# Autodesk Inventor assembly: Cover
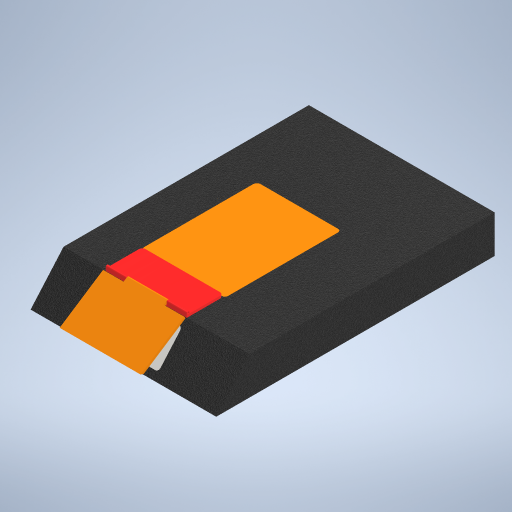
[picture p0: Inventor's stored thumbnail of the model, 512x512]
Saved by Autodesk Inventor 2023 (Build 270158000, 158)
## iProperties
Created: 2023-03-08
Part Number: Cover
Document SubType Name: Assembly
Designer: Josh
Author: Josh
## Documents named in this file (5)
- C:\Users\Josh\Documents\HaierFollower\Printed-Upgrades-for-Mingda-Magician-3D-Printers\Protective cover for the screen\Cover.iam
- C:\Users\Josh\Documents\HaierFollower\Printed-Upgrades-for-Mingda-Magician-3D-Printers\Protective cover for the screen\Toolbox cover.ipt
- C:\Users\Josh\Documents\HaierFollower\Printed-Upgrades-for-Mingda-Magician-3D-Printers\Protective cover for the screen\Cover.ipt
- C:\Users\Josh\Documents\HaierFollower\Printed-Upgrades-for-Mingda-Magician-3D-Printers\Protective cover for the screen\Cover2.ipt
- C:\Users\Josh\Documents\HaierFollower\Printed-Upgrades-for-Mingda-Magician-3D-Printers\Protective cover for the screen\3d.ipt
## Components (4 placed, 4 different names)
1. Toolbox cover:1 — Совмещение:1, Совмещение:6, Совмещение:7, Совмещение:8, Совмещение:9, Заподлицо:1, Совмещение:10
2. Cover:1 — Совмещение:1, Совмещение:4, Совмещение:5, Совмещение:11, Совмещение:12
3. Cover2:1 — Совмещение:4, Совмещение:5
4. 3d:1 — Совмещение:9, Заподлицо:1, Совмещение:10, Совмещение:11, Совмещение:12
## Relationships (11: Mate 10, Flush 1)
- Совмещение:1 [Mate]: Toolbox cover:1 ↔ Cover:1
- Совмещение:4 [Mate]: Cover:1 ↔ Cover2:1
- Совмещение:5 [Mate] (0.25 mm): Cover:1 ↔ Cover2:1
- Совмещение:6 [Mate]: Toolbox cover:1
- Совмещение:7 [Mate]: Toolbox cover:1
- Совмещение:8 [Mate]: Toolbox cover:1
- Совмещение:9 [Mate]: Toolbox cover:1 ↔ 3d:1
- Заподлицо:1 [Flush]: Toolbox cover:1 ↔ 3d:1
- Совмещение:10 [Mate]: Toolbox cover:1 ↔ 3d:1
- Совмещение:11 [Mate]: Cover:1 ↔ 3d:1
- Совмещение:12 [Mate] (2 mm): Cover:1 ↔ 3d:1
